# Autodesk Inventor assembly: Drive2
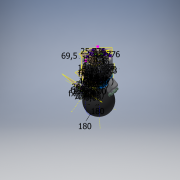
[picture p0: Inventor's stored thumbnail of the model, 180x180]
Saved by Autodesk Inventor 2019.1 (Build 231200000, 200)
## iProperties
Created: 2018-06-30
Part Number: Drive2
Material: Generisch
Document SubType Name: Assembly
Designer: JochenAlt
Author: JochenAlt
## Documents named in this file (9)
- D:\Projects\Ondine\CAD\Drive.iam
- D:\Projects\Ondine\CAD\Sphere.ipt
- D:\Projects\Ondine\CAD\DriveChain.iam
- D:\Projects\Ondine\CAD\Spindle\SpindleWithGear.ipt
- D:\Projects\Ondine\CAD\Spindle\Spindle.ipt
- D:\Projects\Ondine\CAD\Bearings\W 61700 X-2RS1.iam
- D:\Projects\Ondine\CAD\SpindleMotor.iam
- D:\Projects\Ondine\CAD\PCB\ControllerPCBHolder.ipt
- D:\Projects\Ondine\CAD\PCB\MotorController.ipt
## Components (16 placed, 7 different names)
1. Sphere:1 — Passend:38, Passend:61
2. DriveChain:1 [sub-assembly] — Passend:60, Passend:61, Passend:91, Passend:95, Passend:98, Passend:102, Passend:103, Passend:104, Passend:105
3. DriveChain:2 [sub-assembly] — Passend:84, Passend:87, Passend:95, Passend:97, Passend:99, Passend:109
4. DriveChain:3 [sub-assembly] — Passend:89, Passend:93, Passend:97, Passend:98, Passend:103, Passend:104
5. Spindle:1 — Passend:66, Passend:70, Passend:72, Passend:77, Fluchtend:1
6. Spindle:2 — Passend:67, Passend:69, Passend:75, Passend:76, Passend:93
7. Spindle:3 — Passend:73, Passend:101, Passend:102
8. W 61700 X-2RS1:1 [sub-assembly] — Passend:66, Passend:70
9. W 61700 X-2RS1:2 [sub-assembly]
10. W 61700 X-2RS1:3 [sub-assembly] — Passend:67, Passend:69
11. W 61700 X-2RS1:4 [sub-assembly] — Passend:72, Passend:77, Passend:87, Passend:109
12. W 61700 X-2RS1:5 [sub-assembly] — Passend:75, Passend:76, Passend:89
13. W 61700 X-2RS1:6 [sub-assembly] — Passend:73, Passend:91, Passend:101
14. SpindleMotor:1 [sub-assembly] — Passend:84, Fluchtend:1
15. ControllerPCBHolder:1 — Passend:99, Passend:105, Passend:106, Passend:107, Passend:108
16. MotorController:1 — Passend:106, Passend:107, Passend:108
## Relationships (31: Mate 30, Flush 1)
- Passend:38 [Mate]: Sphere:1
- Passend:60 [Mate]: DriveChain:1
- Passend:61 [Mate] (89 mm): Sphere:1 ↔ DriveChain:1
- Passend:66 [Mate]: Spindle:1 ↔ W 61700 X-2RS1:1
- Passend:67 [Mate]: Spindle:2 ↔ W 61700 X-2RS1:3
- Passend:69 [Mate]: Spindle:2 ↔ W 61700 X-2RS1:3
- Passend:70 [Mate]: Spindle:1 ↔ W 61700 X-2RS1:1
- Passend:72 [Mate]: Spindle:1 ↔ W 61700 X-2RS1:4
- Passend:73 [Mate]: Spindle:3 ↔ W 61700 X-2RS1:6
- Passend:75 [Mate]: Spindle:2 ↔ W 61700 X-2RS1:5
- Passend:76 [Mate]: Spindle:2 ↔ W 61700 X-2RS1:5
- Passend:77 [Mate]: Spindle:1 ↔ W 61700 X-2RS1:4
- Passend:84 [Mate]: DriveChain:2 ↔ SpindleMotor:1
- Fluchtend:1 [Flush]: Spindle:1 ↔ SpindleMotor:1
- Passend:87 [Mate]: DriveChain:2 ↔ W 61700 X-2RS1:4
- Passend:89 [Mate]: DriveChain:3 ↔ W 61700 X-2RS1:5
- Passend:91 [Mate]: DriveChain:1 ↔ W 61700 X-2RS1:6
- Passend:93 [Mate]: DriveChain:3 ↔ Spindle:2
- Passend:95 [Mate]: DriveChain:1 ↔ DriveChain:2
- Passend:97 [Mate]: DriveChain:2 ↔ DriveChain:3
- Passend:98 [Mate]: DriveChain:1 ↔ DriveChain:3
- Passend:99 [Mate]: DriveChain:2 ↔ ControllerPCBHolder:1
- Passend:101 [Mate]: Spindle:3 ↔ W 61700 X-2RS1:6
- Passend:102 [Mate]: DriveChain:1 ↔ Spindle:3
- Passend:103 [Mate]: DriveChain:1 ↔ DriveChain:3
- Passend:104 [Mate]: DriveChain:1 ↔ DriveChain:3
- Passend:105 [Mate]: DriveChain:1 ↔ ControllerPCBHolder:1
- Passend:106 [Mate]: ControllerPCBHolder:1 ↔ MotorController:1
- Passend:107 [Mate]: ControllerPCBHolder:1 ↔ MotorController:1
- Passend:108 [Mate]: ControllerPCBHolder:1 ↔ MotorController:1
- Passend:109 [Mate]: DriveChain:2 ↔ W 61700 X-2RS1:4
